# Autodesk Inventor assembly: ensamblaje_dedo
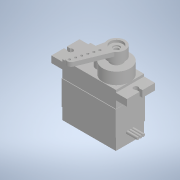
[picture p0: Inventor's stored thumbnail of the model, 180x180]
Saved by Autodesk Inventor 2020 (Build 240168000, 168)
## iProperties
Created: 2021-07-21
Part Number: ensamblaje_dedo
Document SubType Name: Assembly
Designer: chalo
Author: chalo
## Documents named in this file (3)
- C:\Users\chalo\OneDrive\Documents\GitHub\Interfaces-Biomedicas-2021\Gonzalo Palarea\Inventor\ensamblaje_dedo.iam
- C:\Users\chalo\OneDrive\Documents\GitHub\Interfaces-Biomedicas-2021\Gonzalo Palarea\Inventor\referencias\MG90_Rebuild.ipt
- C:\Users\chalo\OneDrive\Documents\GitHub\Interfaces-Biomedicas-2021\Gonzalo Palarea\Inventor\referencias\Arm01.ipt
## Components (2 placed, 2 different names)
1. MG90_Rebuild:1 — Insert:1
2. Arm01:1 — Insert:1
## Relationships (1: Insert 1)
- Insert:1: MG90_Rebuild:1 ↔ Arm01:1
